# Autodesk Inventor assembly: CAM13
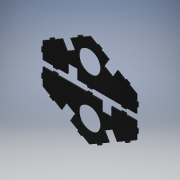
[picture p0: Inventor's stored thumbnail of the model, 180x180]
Saved by Autodesk Inventor 2017 (Build 210142000, 142)
## iProperties
Created: 2019-06-07
Part Number: CAM13
Document SubType Name: Assembly
Designer: Dell
Author: Dell
## Documents named in this file (2)
- C:\Users\Dell\Documents\GitHub\tr2\Body 2.0\CAM13.iam
- C:\Users\Dell\Documents\GitHub\tr2\Body 2.0\BA19.ipt
## Components (2 placed, 1 different names)
1. BA19:1 — Mate:1, Angle:1, Flush:1
2. BA19:2 — Mate:2, Angle:1, Flush:1
## Relationships (4: Mate 2, Angle 1, Flush 1)
- Mate:1: BA19:1
- Mate:2: BA19:2
- Angle:1 (180 deg): BA19:1 ↔ BA19:2
- Flush:1: BA19:1 ↔ BA19:2
